# Autodesk Inventor assembly: Motor_ZSB
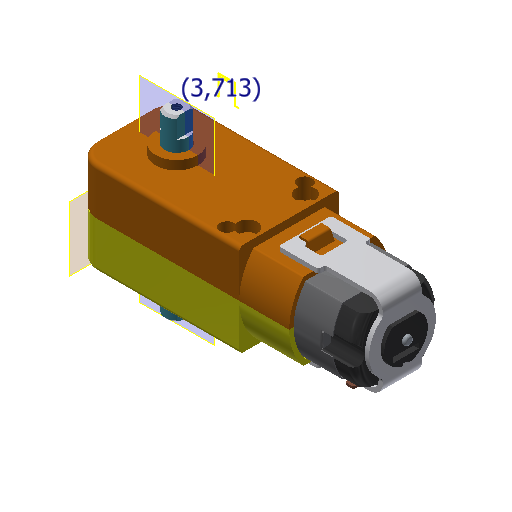
[picture p0: Inventor's stored thumbnail of the model, 512x512]
Saved by Autodesk Inventor 2025.1 (Build 291241000, 241)
## iProperties
Created: 2022-10-31
Part Number: Motor_ZSB
Material: Generisch
Document SubType Name: Assembly
Designer: RP
Author: RP
## Documents named in this file (11)
- C:\Users\Erik\Erik\Hochschule\3. Semester\CAD\CAD-Paspa\Useless Box\_Useless_Box\Motor_ZSB.iam
- C:\Users\Erik\Erik\Hochschule\3. Semester\CAD\CAD-Paspa\Useless Box\_Useless_Box\Motor_Unterseite.ipt
- C:\Users\Erik\Erik\Hochschule\3. Semester\CAD\CAD-Paspa\Useless Box\_Useless_Box\Motor.ipt
- C:\Users\Erik\Erik\Hochschule\3. Semester\CAD\CAD-Paspa\Useless Box\_Useless_Box\Motor_Achse.ipt
- C:\Users\Erik\Erik\Hochschule\3. Semester\CAD\CAD-Paspa\Useless Box\_Useless_Box\Motor_Ausgangswelle.ipt
- C:\Users\Erik\Erik\Hochschule\3. Semester\CAD\CAD-Paspa\Useless Box\_Useless_Box\Motor_Oberseite.ipt
- C:\Users\Erik\Erik\Hochschule\3. Semester\CAD\CAD-Paspa\Useless Box\_Useless_Box\Motor_Sicherungsblech.ipt
- C:\Users\Erik\Erik\Hochschule\3. Semester\CAD\CAD-Paspa\Useless Box\_Useless_Box\Motor_Stirnradpaar_2_3.ipt
- C:\Users\Erik\Erik\Hochschule\3. Semester\CAD\CAD-Paspa\Useless Box\_Useless_Box\Motor_Stirnradpaar_3_4.ipt
- C:\Users\Erik\Erik\Hochschule\3. Semester\CAD\CAD-Paspa\Useless Box\_Useless_Box\Motor_Tellerrad.ipt
- C:\Users\Erik\Erik\Hochschule\3. Semester\CAD\CAD-Paspa\Useless Box\_Useless_Box\Motor_Schraube.ipt
## Components (11 placed, 10 different names)
1. Motor_Unterseite:1 — Passend:1, Fluchtend:1, Passend:2, Einfügen:1, Einfügen:2, Einfügen:3, Einfügen:5, Winkel:1, Passend:4, Winkel:2, Einfügen:10, Einfügen:11
2. Motor_Ausgangswelle:1 — Einfügen:1, Einfügen:4, Passend:3, Winkel:5
3. Motor_Achse:1 — Einfügen:2
4. Motor_Stirnradpaar_3_4:1 — Einfügen:3, Einfügen:6
5. Motor_Stirnradpaar_2_3:1 — Einfügen:4
6. Motor:1 — Einfügen:5, Winkel:1, Einfügen:7, Winkel:3, Winkel:5
7. Motor_Tellerrad:1 — Einfügen:6
8. Motor_Oberseite:1 — Passend:3, Passend:4, Winkel:2
9. Motor_Schraube:1 — Einfügen:10, Winkel:4
10. Motor_Schraube:2 — Einfügen:11
11. Motor_Sicherungsblech:1 — Einfügen:7, Winkel:3, Winkel:4
## Relationships (19: Insert 9, Angle 5, Mate 4, Flush 1)
- Passend:1 [Mate]: Motor_Unterseite:1
- Fluchtend:1 [Flush]: Motor_Unterseite:1
- Passend:2 [Mate]: Motor_Unterseite:1
- Einfügen:1 [Insert]: Motor_Unterseite:1 ↔ Motor_Ausgangswelle:1
- Einfügen:2 [Insert]: Motor_Unterseite:1 ↔ Motor_Achse:1
- Einfügen:3 [Insert]: Motor_Unterseite:1 ↔ Motor_Stirnradpaar_3_4:1
- Einfügen:4 [Insert]: Motor_Ausgangswelle:1 ↔ Motor_Stirnradpaar_2_3:1
- Einfügen:5 [Insert]: Motor_Unterseite:1 ↔ Motor:1
- Winkel:1 [Angle] (0 deg): Motor_Unterseite:1 ↔ Motor:1
- Einfügen:6 [Insert] (0.3 mm): Motor_Stirnradpaar_3_4:1 ↔ Motor_Tellerrad:1
- Passend:3 [Mate]: Motor_Ausgangswelle:1 ↔ Motor_Oberseite:1
- Passend:4 [Mate]: Motor_Unterseite:1 ↔ Motor_Oberseite:1
- Winkel:2 [Angle] (0 deg): Motor_Unterseite:1 ↔ Motor_Oberseite:1
- Einfügen:7 [Insert]: Motor:1 ↔ Motor_Sicherungsblech:1
- Winkel:3 [Angle] (180 deg): Motor:1 ↔ Motor_Sicherungsblech:1
- Einfügen:10 [Insert]: Motor_Unterseite:1 ↔ Motor_Schraube:1
- Winkel:4 [Angle] (0 deg): Motor_Schraube:1 ↔ Motor_Sicherungsblech:1
- Einfügen:11 [Insert]: Motor_Unterseite:1 ↔ Motor_Schraube:2
- Winkel:5 [Angle] (0.2 deg): Motor_Ausgangswelle:1 ↔ Motor:1
